# Autodesk Inventor assembly: wheel
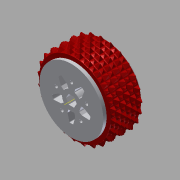
[picture p0: Inventor's stored thumbnail of the model, 180x180]
Saved by Autodesk Inventor 2013 (Build 170138000, 138)
## iProperties
Created: 2013-04-30
Part Number: wheel
Document SubType Name: Assembly
Designer: grtstudent
Author: grtstudent
## Documents named in this file (3)
- C:\Users\grtstudent\Desktop\Mark 6 Final Preseason\Base (2013)\Wheels\wheel.iam
- C:\Users\grtstudent\Desktop\Mark 6 Final Preseason\Base (2013)\Wheels\Wheel Hub.ipt
- C:\Users\grtstudent\Desktop\Mark 6 Final Preseason\Base (2013)\Wheels\Wheel Tread Test 2.ipt
## Components (3 placed, 2 different names)
1. Wheel Hub:1 — Mate:1, Mate:2, Flush:1, Mate:4
2. Wheel Hub:2 — Mate:1, Mate:2, Flush:1, Mate:3, Mate:5
3. Wheel Tread Test 2:1 — Mate:3, Mate:4, Mate:5
## Relationships (6: Mate 5, Flush 1)
- Mate:1: Wheel Hub:1 ↔ Wheel Hub:2
- Mate:2: Wheel Hub:1 ↔ Wheel Hub:2
- Flush:1: Wheel Hub:1 ↔ Wheel Hub:2
- Mate:3: Wheel Hub:2 ↔ Wheel Tread Test 2:1
- Mate:4: Wheel Hub:1 ↔ Wheel Tread Test 2:1
- Mate:5: Wheel Hub:2 ↔ Wheel Tread Test 2:1
